# Autodesk Inventor assembly: AM14U3 Wide Half
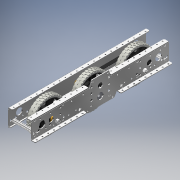
[picture p0: Inventor's stored thumbnail of the model, 180x180]
Saved by Autodesk Inventor 2017 (Build 210142000, 142)
## iProperties
Created: 2017-01-12
Part Number: AM14U3 Wide Half
Document SubType Name: Assembly
Designer: Ben
Author: Ben
Revision Number: ANY
## Documents named in this file (8)
- C:\Users\Ben\Desktop\Projects\2017 Robot\Frame\AM14U3 Wide Half.iam
- C:\Users\Ben\Desktop\Projects\2017 Robot\Frame\AM14U3 Wide Frame Half.iam
- C:\Users\Ben\Desktop\Projects\2017 Robot\Frame\FR8ZZ Hex Bearing.ipt
- C:\Users\Ben\Desktop\Projects\2017 Robot\Frame\6 HiGrip with hub and double pulley.iam
- C:\Users\Ben\Desktop\Projects\2017 Robot\Frame\6 HiGrip with bearings, pulleys and spacers.iam
- C:\Users\Ben\Desktop\Projects\2017 Robot\Frame\375-16 x 4.25 Hex Bolt_HFBOLT 0.375-16x2.5x1-C.ipt
- C:\Users\Ben\Desktop\Projects\2017 Robot\Frame\375-16 Lock Nut_91831A127.ipt
- C:\Users\Ben\Desktop\Projects\2017 Robot\Frame\am-2704 600-5M-15 Timing Belt.ipt
## Components (10 placed, 10 different names)
1. AM14U3 Wide Frame Half_9 [sub-assembly] — Insert:1
2. FR8ZZ Hex Bearing_10 — Insert:1
3. 6 HiGrip with hub and double pulley_11 [sub-assembly]
4. 6 HiGrip with bearings, pulleys and spacers_12 [sub-assembly]
5. 6 HiGrip with bearings, pulleys and spacers_13 [sub-assembly]
6. 375-16 x 4.25 Hex Bolt_HFBOLT 0.375-16x2.5x1-C_14
7. 375-16 Lock Nut_91831A127_15
8. 375-16 Lock Nut_91831A127_16
9. am-2704 600-5M-15 Timing Belt_17
10. am-2704 600-5M-15 Timing Belt_18
## Relationships (1: Insert 1)
- Insert:1: AM14U3 Wide Frame Half_9 ↔ FR8ZZ Hex Bearing_10
